# Autodesk Inventor assembly: mg996r_servo_frame_with_axis
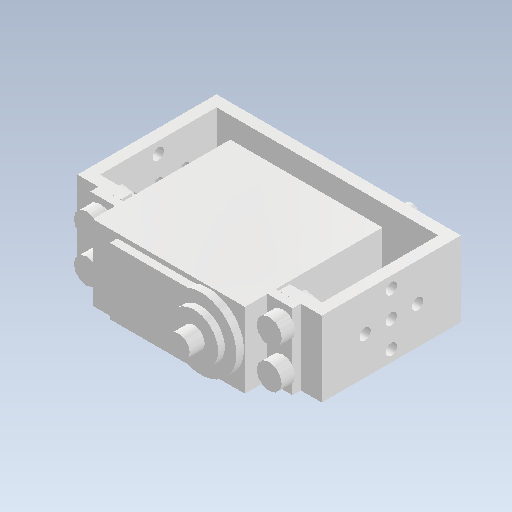
[picture p0: Inventor's stored thumbnail of the model, 512x512]
Saved by Autodesk Inventor 2021.4 (Build 254397000, 397)
## iProperties
Created: 2022-07-24
Part Number: mg996r_servo_frame_with_axis
Document SubType Name: Assembly
Designer: isamu
Author: isamu
## Documents named in this file (4)
- D:\personal_projects\robot\inventor\2021_matlab_compat\mg996r_servo_frame_with_axis.iam
- D:\personal_projects\robot\inventor\2021_matlab_compat\mg996r_servo_frame.iam
- D:\personal_projects\robot\exports\screws\m4x12.ipt
- D:\personal_projects\robot\exports\screws\m4 nuts.ipt
## Components (3 placed, 3 different names)
1. mg996r_servo_frame:1 [sub-assembly] — Insert:1, Insert:2
2. m4x12:1 — Insert:1
3. m4 nuts:1 — Insert:2
## Relationships (2: Insert 2)
- Insert:1: mg996r_servo_frame:1 ↔ m4x12:1
- Insert:2: mg996r_servo_frame:1 ↔ m4 nuts:1
